# Autodesk Inventor assembly: Assembly_BRIDA
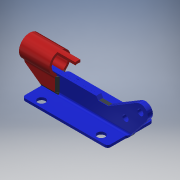
[picture p0: Inventor's stored thumbnail of the model, 180x180]
Saved by Autodesk Inventor 2018 (Build 220112000, 112)
## iProperties
Created: 2018-10-25
Part Number: Assembly_BRIDA
Document SubType Name: Weldment
Designer: Isaac
Weld Material: Iron, Gray
Author: Isaac
## Documents named in this file (4)
- Y:\BRIDA DE APRIETE\Assembly_BRIDA.iam
- Y:\BRIDA DE APRIETE\Part1_IZQ.ipt
- Y:\BRIDA DE APRIETE\Part1_DER.ipt
- Y:\BRIDA DE APRIETE\Part2.ipt
## Components (3 placed, 3 different names)
1. Part1_IZQ:1 — Mate:1, Mate:2, Mate:3, Mate:4, Mate:5
2. Part1_DER:1 — Mate:1, Mate:2
3. Part2:1 — Mate:3, Mate:4, Mate:5
## Relationships (5: Mate 5)
- Mate:1: Part1_IZQ:1 ↔ Part1_DER:1
- Mate:2: Part1_IZQ:1 ↔ Part1_DER:1
- Mate:3: Part1_IZQ:1 ↔ Part2:1
- Mate:4 (-15 mm): Part1_IZQ:1 ↔ Part2:1
- Mate:5 (2.5 mm): Part1_IZQ:1 ↔ Part2:1
